# Autodesk Inventor assembly: 574335 SMT-8M-A-PS-24V-E-2,5-OE
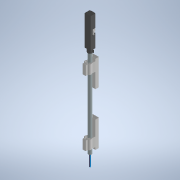
[picture p0: Inventor's stored thumbnail of the model, 180x180]
Saved by Autodesk Inventor 2021 (Build 250183000, 183)
## iProperties
Category: PARTsolutions
Company: FESTO
Created: 2026-04-08
Part Number: 574335 SMT-8M-A-PS-24V-E-2,5-OE
Catalog Web Link: www.3dfindit.com
Description: SMT-8M-A-proximity sensor
Vendor: FESTO
Document SubType Name: Assembly
Designer: psAdmin
Manufacturer: FESTO
Mass: 29.1 g
Surface Area: 36.9113 cm^2
Volume: 1.70669 cm^3
Density: 17.0506 g/cm^3
Title: 574335 SMT-8M-A-PS-24V-E-2,5-OE
Author: Cadenas PARTsolutions
Comments: proximity sensor
PSOL_IDENT_0: {ATYP=ASSISTANT},{DATA=script=$CADENAS_DATA/23d-libs/festo/webfesto.vbb&M_FAMILY=SMT&M_GROUP=01&M_PA
PSOL_IDENT_1: RTNO=574335&IDCODE1=SMT-8M-A-PS-24V-E-25-OE&IDCODE2=&customer_number_cns=&MATES=1&LOD=HI&LOCKERP=0&S
PSOL_IDENT_2: INGLEPART=1}
NB: 574335 SMT-8M-A-PS-24V-E-2,5-OE
NN: SMT-8M-A
NT: proximity sensor
NBSYN: $TNR. $TYP.
LINA: 574335 SMT-8M-A-PS-24V-E-2,5-OE
CATALOG: Festo
TNR: 574335
TYP: SMT-8M-A-PS-24V-E-2,5-OE
CNSMASSEXACT: 0.0291
GTIN: 4052568103101
REACH: Yes
REACHSVHC: Yes
REACHHAZSUBS: 7439-92-1
REACHVALDATE: 05.03.2025
SUPPLIER: FESTO
ARTICLENO: 574335 SMT-8M-A-PS-24V-E-2,5-OE
BOMINFO: 574335 SMT-8M-A-PS-24V-E-2,5-OE
CREATOR: CADENAS GmbH
## Documents named in this file (3)
- e:\temp\worker_COMMON_40\temp\tmp_8940_54_pwRLH\format_0\574335 SMT-8M-A-PS-24V-E-2,5-OE.iam
- e:\temp\worker_COMMON_40\temp\tmp_8940_54_pwRLH\format_0\574333 SMT-8M-A-1---OE---(part).ipt
- e:\temp\worker_COMMON_40\temp\tmp_8940_54_pwRLH\format_0\1247168 ASCF-M-23-S DM 2_1-3_4.ipt
## Components (3 placed, 2 different names)
1. 574333 SMT-8M-A-1---OE---(part):1 — ASCF1_XY@1 <-> KTN_XY@2, ASCF1_Z@1 <-> KTN_Z@2, ASCF1_YZ@1 <-> KTN_YZ@2, ASCF2_XY@1 <-> KTN_XY@3, ASCF2_Z@1 <-> KTN_Z@3, ASCF2_YZ@1 <-> KTN_YZ@3
2. 1247168 ASCF-M-23-S DM 2_1-3_4:1 — ASCF1_XY@1 <-> KTN_XY@2, ASCF1_Z@1 <-> KTN_Z@2, ASCF1_YZ@1 <-> KTN_YZ@2
3. 1247168 ASCF-M-23-S DM 2_1-3_4:2 — ASCF2_XY@1 <-> KTN_XY@3, ASCF2_Z@1 <-> KTN_Z@3, ASCF2_YZ@1 <-> KTN_YZ@3
## Relationships (6: Mate 4, Angle 2)
- ASCF1_XY@1 <-> KTN_XY@2 [Mate]: 574333 SMT-8M-A-1---OE---(part):1 ↔ 1247168 ASCF-M-23-S DM 2_1-3_4:1
- ASCF1_Z@1 <-> KTN_Z@2 [Mate]: 574333 SMT-8M-A-1---OE---(part):1 ↔ 1247168 ASCF-M-23-S DM 2_1-3_4:1
- ASCF1_YZ@1 <-> KTN_YZ@2 [Angle] (0 deg): 574333 SMT-8M-A-1---OE---(part):1 ↔ 1247168 ASCF-M-23-S DM 2_1-3_4:1
- ASCF2_XY@1 <-> KTN_XY@3 [Mate]: 574333 SMT-8M-A-1---OE---(part):1 ↔ 1247168 ASCF-M-23-S DM 2_1-3_4:2
- ASCF2_Z@1 <-> KTN_Z@3 [Mate]: 574333 SMT-8M-A-1---OE---(part):1 ↔ 1247168 ASCF-M-23-S DM 2_1-3_4:2
- ASCF2_YZ@1 <-> KTN_YZ@3 [Angle] (180 deg): 574333 SMT-8M-A-1---OE---(part):1 ↔ 1247168 ASCF-M-23-S DM 2_1-3_4:2
